# Autodesk Inventor assembly: MotorWithAxis
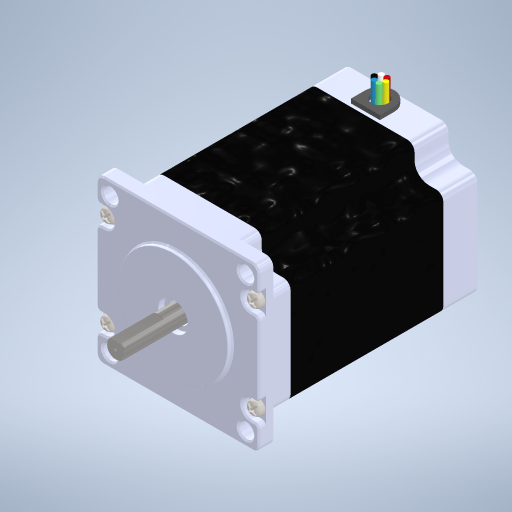
[picture p0: Inventor's stored thumbnail of the model, 512x512]
Saved by Autodesk Inventor 2023 (Build 270158000, 158)
## iProperties
Created: 2024-02-07
Part Number: MotorWithAxis
Document SubType Name: Assembly
Designer: victo
Author: victo
## Documents named in this file (3)
- C:\Users\victo\Documents\ball-balancing-digital-twin\Mechanics\CAD\MotorWithAxis.iam
- C:\Users\victo\Documents\ball-balancing-digital-twin\Mechanics\CAD\Step Motor Nema AK23 - 15kg.ipt
- C:\Users\victo\Documents\ball-balancing-digital-twin\Mechanics\CAD\motorAxis.ipt
## Components (2 placed, 2 different names)
1. Step Motor Nema AK23 - 15kg:1 — Mate:1, Flush:1
2. motorAxis:1 — Mate:1, Flush:1
## Relationships (2: Mate 1, Flush 1)
- Mate:1: Step Motor Nema AK23 - 15kg:1 ↔ motorAxis:1
- Flush:1: Step Motor Nema AK23 - 15kg:1 ↔ motorAxis:1
